# Autodesk Inventor assembly: Assembly2
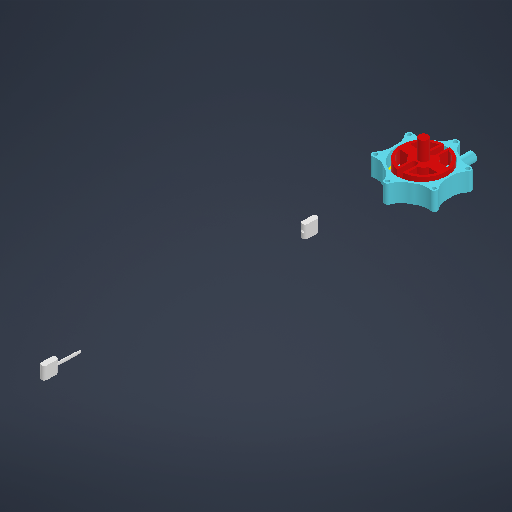
[picture p0: Inventor's stored thumbnail of the model, 512x512]
Saved by Autodesk Inventor 2025.3 (Build 293356000, 356)
## iProperties
Created: 2025-10-08
Part Number: Assembly2
Document SubType Name: Assembly
Designer: sophi
Author: sophi
## Documents named in this file (7)
- C:\Users\sophi\OneDrive - Universidad de los andes\Documentos\1 Universidad\5 Semestre\Herramientas\Huron-Hudson\Vane Engine\Vane\Assembly2.iam
- C:\Users\sophi\OneDrive - Universidad de los andes\Documentos\1 Universidad\5 Semestre\Herramientas\Huron-Hudson\Vane Engine\Vane\intermo.ipt
- C:\Users\sophi\OneDrive - Universidad de los andes\Documentos\1 Universidad\5 Semestre\Herramientas\Huron-Hudson\Vane Engine\Vane\paletas - copia.ipt
- C:\Users\sophi\OneDrive - Universidad de los andes\Documentos\1 Universidad\5 Semestre\Herramientas\Huron-Hudson\Vane Engine\Vane\paletas.ipt
- C:\Users\sophi\OneDrive - Universidad de los andes\Documentos\1 Universidad\5 Semestre\Herramientas\Huron-Hudson\Vane Engine\Vane\rodamiento.ipt
- C:\Users\sophi\OneDrive - Universidad de los andes\Documentos\1 Universidad\5 Semestre\Herramientas\Huron-Hudson\Vane Engine\Vane\tapa.ipt
- C:\Users\sophi\OneDrive - Universidad de los andes\Documentos\1 Universidad\5 Semestre\Herramientas\Huron-Hudson\Vane Engine\Vane\carcaza motor.ipt
## Components (6 placed, 6 different names)
1. intermo:1 — Mate:5, Mate:9
2. paletas - copia:1 — Mate:1, Mate:5, Mate:7
3. paletas:1 — Mate:1
4. rodamiento:1 — Mate:6, Mate:7, Mate:8, Mate:9
5. tapa:1 — Flush:4, Flush:5, Mate:3
6. carcaza motor:1 — Flush:1, Flush:2, Flush:3, Flush:4, Flush:5, Mate:3, Mate:6, Mate:8
## Relationships (12: Mate 7, Flush 5)
- Flush:1: carcaza motor:1
- Flush:2: carcaza motor:1
- Flush:3: carcaza motor:1
- Mate:1: paletas - copia:1 ↔ paletas:1
- Flush:4: tapa:1 ↔ carcaza motor:1
- Flush:5: tapa:1 ↔ carcaza motor:1
- Mate:3: tapa:1 ↔ carcaza motor:1
- Mate:5: intermo:1 ↔ paletas - copia:1
- Mate:6: rodamiento:1 ↔ carcaza motor:1
- Mate:7: paletas - copia:1 ↔ rodamiento:1
- Mate:8: rodamiento:1 ↔ carcaza motor:1
- Mate:9: intermo:1 ↔ rodamiento:1
